# Autodesk Inventor assembly: BeamAssembly
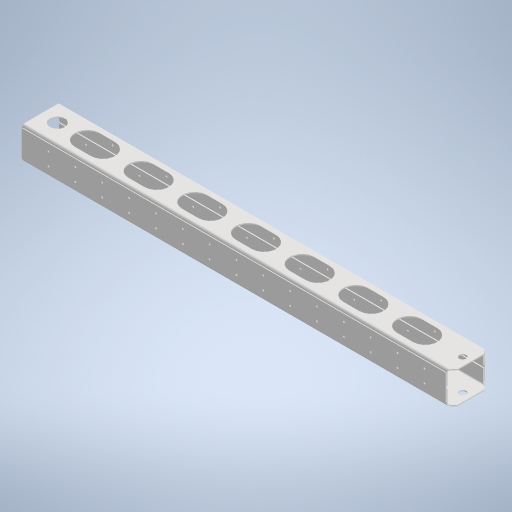
[picture p0: Inventor's stored thumbnail of the model, 512x512]
Saved by Autodesk Inventor 2023 (Build 270158000, 158)
## iProperties
Created: 2023-05-02
Part Number: BeamAssembly
Document SubType Name: Assembly
Designer: emila
Author: emila
## Documents named in this file (4)
- C:\Users\emila\Documents\GitHub\MER_MiniProject\3D Models\Beam\BeamAssembly.iam
- C:\Users\emila\Documents\GitHub\MER_MiniProject\3D Models\Beam\beam.ipt
- C:\Users\emila\Documents\GitHub\MER_MiniProject\3D Models\Beam\connectionPlate.ipt
- C:\Users\emila\Documents\GitHub\MER_MiniProject\3D Models\Cylinder\193993 DSNU-40-300-P-A---(300PA---00--0-------0).iam
## Components (5 placed, 3 different names)
1. beam:1 — Flush:1, Flush:2, Mate:5
2. beam:2 — Flush:1, Flush:2, Mate:1, Mate:2, Mate:3, Mate:4
3. connectionPlate:1 — Mate:1, Mate:3, Mate:5
4. connectionPlate:2 — Mate:2, Mate:4
5. 193993 DSNU-40-300-P-A---(300PA---00--0-------0):1 [sub-assembly]
## Relationships (7: Mate 5, Flush 2)
- Flush:1: beam:1 ↔ beam:2
- Flush:2: beam:1 ↔ beam:2
- Mate:1: beam:2 ↔ connectionPlate:1
- Mate:2: beam:2 ↔ connectionPlate:2
- Mate:3: beam:2 ↔ connectionPlate:1
- Mate:4: beam:2 ↔ connectionPlate:2
- Mate:5: beam:1 ↔ connectionPlate:1
